# Autodesk Inventor assembly: ONDERPLAAT
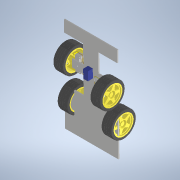
[picture p0: Inventor's stored thumbnail of the model, 180x180]
Saved by Autodesk Inventor 2022 (Build 260153000, 153)
## iProperties
Created: 2021-12-16
Part Number: ONDERPLAAT
Document SubType Name: Assembly
Designer: keemi
Author: keemi
## Documents named in this file (6)
- C:\Users\keemi\OneDrive\Bureaublad\repo's\projecten\Auto\modellen\inventor\auto moddel\ONDERPLAAT.iam
- C:\Users\keemi\OneDrive\Bureaublad\repo's\projecten\Auto\modellen\inventor\auto moddel\onderkant.ipt
- C:\Users\keemi\OneDrive\Bureaublad\repo's\projecten\Auto\modellen\inventor\geared-dc-motor-for-arduino-applications-1.snapshot.2\Hobi - Motor DC 1.ipt
- C:\Users\keemi\OneDrive\Bureaublad\repo's\projecten\Auto\modellen\inventor\wheel-arduino-1.snapshot.2\Wheel ALL.ipt
- C:\Users\keemi\OneDrive\Bureaublad\repo's\projecten\Auto\modellen\inventor\SG90\SG90 v1.ipt
- C:\Users\keemi\OneDrive\Bureaublad\repo's\projecten\Auto\modellen\inventor\auto moddel\STUURAS.ipt
## Components (10 placed, 5 different names)
1. onderkant:1 — Mate:9, Flush:1, Mate:10, Flush:3, Flush:4, Mate:11, Flush:5, Flush:6, Mate:16, Mate:17
2. Hobi - Motor DC 1:1 — Mate:1, Mate:2, Mate:10, Flush:2, Flush:4
3. Wheel ALL:1 — Mate:1, Mate:2
4. Hobi - Motor DC 1:2 — Mate:9, Flush:1, Flush:2, Flush:3
5. Wheel ALL:2
6. SG90 v1:1 — Mate:11, Flush:5, Flush:6
7. STUURAS:1 — Mate:12, Mate:13, Mate:16
8. Wheel ALL:3 — Mate:12, Mate:13
9. STUURAS:2 — Mate:17
10. Wheel ALL:4
## Relationships (19: Mate 13, Flush 6)
- Mate:1: Hobi - Motor DC 1:1 ↔ Wheel ALL:1
- Mate:2: Hobi - Motor DC 1:1 ↔ Wheel ALL:1
- [Mate]: Hobi - Motor DC 1:2 ↔ Wheel ALL:2
- [Mate]: Hobi - Motor DC 1:2 ↔ Wheel ALL:2
- Mate:9: onderkant:1 ↔ Hobi - Motor DC 1:2
- Flush:1 (70 mm): onderkant:1 ↔ Hobi - Motor DC 1:2
- Mate:10: onderkant:1 ↔ Hobi - Motor DC 1:1
- Flush:2: Hobi - Motor DC 1:1 ↔ Hobi - Motor DC 1:2
- Flush:3 (30 mm): onderkant:1 ↔ Hobi - Motor DC 1:2
- Flush:4 (30 mm): onderkant:1 ↔ Hobi - Motor DC 1:1
- Mate:11: onderkant:1 ↔ SG90 v1:1
- Flush:5 (70 mm): onderkant:1 ↔ SG90 v1:1
- Flush:6 (65 mm): onderkant:1 ↔ SG90 v1:1
- Mate:12: STUURAS:1 ↔ Wheel ALL:3
- Mate:13: STUURAS:1 ↔ Wheel ALL:3
- [Mate]: STUURAS:2 ↔ Wheel ALL:4
- [Mate]: STUURAS:2 ↔ Wheel ALL:4
- Mate:16: onderkant:1 ↔ STUURAS:1
- Mate:17: onderkant:1 ↔ STUURAS:2
## Named parameters: d2_d0 = 0 mm, d3_d1 = 0 mm, d24_d22 = 0 mm, d25_d23 = 0 mm
